# Autodesk Inventor assembly: Assembly1
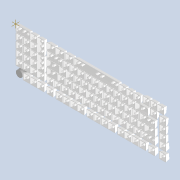
[picture p0: Inventor's stored thumbnail of the model, 180x180]
Saved by Autodesk Inventor 2021 (Build 250183000, 183)
## iProperties
Created: 2021-12-04
Part Number: Assembly1
Document SubType Name: Assembly
Designer: Matthew Flooks
Author: Matthew Flooks
## Documents named in this file (106)
- C:\Users\Matthew Flooks\Documents\GitHub\QEX103-PCB\3D Model\Assembly1.iam
- C:\Users\Matthew Flooks\Documents\GitHub\QEX103-PCB\3D Model\Layout.ipt
- C:\Users\Matthew Flooks\Documents\GitHub\QEX103-PCB\3D Model\KeyCaps\Space.ipt
- C:\Users\Matthew Flooks\Documents\GitHub\QEX103-PCB\3D Model\KeyCaps\Menu.ipt
- C:\Users\Matthew Flooks\Documents\GitHub\QEX103-PCB\3D Model\KeyCaps\CtrlRight.ipt
- C:\Users\Matthew Flooks\Documents\GitHub\QEX103-PCB\3D Model\KeyCaps\AltRight.ipt
- C:\Users\Matthew Flooks\Documents\GitHub\QEX103-PCB\3D Model\KeyCaps\Del.ipt
- C:\Users\Matthew Flooks\Documents\GitHub\QEX103-PCB\3D Model\KeyCaps\Ins.ipt
- C:\Users\Matthew Flooks\Documents\GitHub\QEX103-PCB\3D Model\KeyCaps\F12.ipt
- C:\Users\Matthew Flooks\Documents\GitHub\QEX103-PCB\3D Model\KeyCaps\F11.ipt
- C:\Users\Matthew Flooks\Documents\GitHub\QEX103-PCB\3D Model\KeyCaps\F10.ipt
- C:\Users\Matthew Flooks\Documents\GitHub\QEX103-PCB\3D Model\KeyCaps\F9.ipt
- C:\Users\Matthew Flooks\Documents\GitHub\QEX103-PCB\3D Model\KeyCaps\F8.ipt
- C:\Users\Matthew Flooks\Documents\GitHub\QEX103-PCB\3D Model\KeyCaps\F7.ipt
- C:\Users\Matthew Flooks\Documents\GitHub\QEX103-PCB\3D Model\KeyCaps\F6.ipt
- C:\Users\Matthew Flooks\Documents\GitHub\QEX103-PCB\3D Model\KeyCaps\F5.ipt
- C:\Users\Matthew Flooks\Documents\GitHub\QEX103-PCB\3D Model\KeyCaps\F4.ipt
- C:\Users\Matthew Flooks\Documents\GitHub\QEX103-PCB\3D Model\KeyCaps\F3.ipt
- C:\Users\Matthew Flooks\Documents\GitHub\QEX103-PCB\3D Model\KeyCaps\F2.ipt
- C:\Users\Matthew Flooks\Documents\GitHub\QEX103-PCB\3D Model\KeyCaps\F1.ipt
- C:\Users\Matthew Flooks\Documents\GitHub\QEX103-PCB\3D Model\KeyCaps\Prev.ipt
- C:\Users\Matthew Flooks\Documents\GitHub\QEX103-PCB\3D Model\KeyCaps\Play.ipt
- C:\Users\Matthew Flooks\Documents\GitHub\QEX103-PCB\3D Model\KeyCaps\Next.ipt
- C:\Users\Matthew Flooks\Documents\GitHub\QEX103-PCB\3D Model\KeyCaps\Esc.ipt
- C:\Users\Matthew Flooks\Documents\GitHub\QEX103-PCB\3D Model\KeyCaps\9.ipt
- C:\Users\Matthew Flooks\Documents\GitHub\QEX103-PCB\3D Model\KeyCaps\8.ipt
- C:\Users\Matthew Flooks\Documents\GitHub\QEX103-PCB\3D Model\KeyCaps\7.ipt
- C:\Users\Matthew Flooks\Documents\GitHub\QEX103-PCB\3D Model\KeyCaps\6.ipt
- C:\Users\Matthew Flooks\Documents\GitHub\QEX103-PCB\3D Model\KeyCaps\5.ipt
- C:\Users\Matthew Flooks\Documents\GitHub\QEX103-PCB\3D Model\KeyCaps\4.ipt
- C:\Users\Matthew Flooks\Documents\GitHub\QEX103-PCB\3D Model\KeyCaps\3.ipt
- C:\Users\Matthew Flooks\Documents\GitHub\QEX103-PCB\3D Model\KeyCaps\2.ipt
- C:\Users\Matthew Flooks\Documents\GitHub\QEX103-PCB\3D Model\KeyCaps\1.ipt
- C:\Users\Matthew Flooks\Documents\GitHub\QEX103-PCB\3D Model\KeyCaps\0.ipt
- C:\Users\Matthew Flooks\Documents\GitHub\QEX103-PCB\3D Model\KeyCaps\=.ipt
- C:\Users\Matthew Flooks\Documents\GitHub\QEX103-PCB\3D Model\KeyCaps\~.ipt
- C:\Users\Matthew Flooks\Documents\GitHub\QEX103-PCB\3D Model\KeyCaps\-.ipt
- C:\Users\Matthew Flooks\Documents\GitHub\QEX103-PCB\3D Model\KeyCaps\Backspace.ipt
- C:\Users\Matthew Flooks\Documents\GitHub\QEX103-PCB\3D Model\KeyCaps\Tab.ipt
- C:\Users\Matthew Flooks\Documents\GitHub\QEX103-PCB\3D Model\KeyCaps\Mod.ipt
- C:\Users\Matthew Flooks\Documents\GitHub\QEX103-PCB\3D Model\KeyCaps\ShiftRight.ipt
- C:\Users\Matthew Flooks\Documents\GitHub\QEX103-PCB\3D Model\KeyCaps\CtrlLeft.ipt
- C:\Users\Matthew Flooks\Documents\GitHub\QEX103-PCB\3D Model\KeyCaps\AltLeft.ipt
- C:\Users\Matthew Flooks\Documents\GitHub\QEX103-PCB\3D Model\KeyCaps\Win.ipt
- C:\Users\Matthew Flooks\Documents\GitHub\QEX103-PCB\3D Model\KeyCaps\BackSlash.ipt
- C:\Users\Matthew Flooks\Documents\GitHub\QEX103-PCB\3D Model\KeyCaps\Enter.ipt
- C:\Users\Matthew Flooks\Documents\GitHub\QEX103-PCB\3D Model\KeyCaps\ShiftLeft.ipt
- C:\Users\Matthew Flooks\Documents\GitHub\QEX103-PCB\3D Model\KeyCaps\,.ipt
- C:\Users\Matthew Flooks\Documents\GitHub\QEX103-PCB\3D Model\KeyCaps\..ipt
- C:\Users\Matthew Flooks\Documents\GitHub\QEX103-PCB\3D Model\KeyCaps\B.ipt
- C:\Users\Matthew Flooks\Documents\GitHub\QEX103-PCB\3D Model\KeyCaps\C.ipt
- C:\Users\Matthew Flooks\Documents\GitHub\QEX103-PCB\3D Model\KeyCaps\ForwardSlash.ipt
- C:\Users\Matthew Flooks\Documents\GitHub\QEX103-PCB\3D Model\KeyCaps\M.ipt
- C:\Users\Matthew Flooks\Documents\GitHub\QEX103-PCB\3D Model\KeyCaps\N.ipt
- C:\Users\Matthew Flooks\Documents\GitHub\QEX103-PCB\3D Model\KeyCaps\V.ipt
- C:\Users\Matthew Flooks\Documents\GitHub\QEX103-PCB\3D Model\KeyCaps\X.ipt
- C:\Users\Matthew Flooks\Documents\GitHub\QEX103-PCB\3D Model\KeyCaps\Z.ipt
- C:\Users\Matthew Flooks\Documents\GitHub\QEX103-PCB\3D Model\KeyCaps\A.ipt
- C:\Users\Matthew Flooks\Documents\GitHub\QEX103-PCB\3D Model\KeyCaps\D.ipt
- C:\Users\Matthew Flooks\Documents\GitHub\QEX103-PCB\3D Model\KeyCaps\F.ipt
- C:\Users\Matthew Flooks\Documents\GitHub\QEX103-PCB\3D Model\KeyCaps\G.ipt
- C:\Users\Matthew Flooks\Documents\GitHub\QEX103-PCB\3D Model\KeyCaps\H.ipt
- C:\Users\Matthew Flooks\Documents\GitHub\QEX103-PCB\3D Model\KeyCaps\J.ipt
- C:\Users\Matthew Flooks\Documents\GitHub\QEX103-PCB\3D Model\KeyCaps\K.ipt
- C:\Users\Matthew Flooks\Documents\GitHub\QEX103-PCB\3D Model\KeyCaps\L.ipt
- C:\Users\Matthew Flooks\Documents\GitHub\QEX103-PCB\3D Model\KeyCaps\S.ipt
- C:\Users\Matthew Flooks\Documents\GitHub\QEX103-PCB\3D Model\KeyCaps\'.ipt
- C:\Users\Matthew Flooks\Documents\GitHub\QEX103-PCB\3D Model\KeyCaps\;.ipt
- C:\Users\Matthew Flooks\Documents\GitHub\QEX103-PCB\3D Model\KeyCaps\Q.ipt
- C:\Users\Matthew Flooks\Documents\GitHub\QEX103-PCB\3D Model\KeyCaps\E.ipt
- C:\Users\Matthew Flooks\Documents\GitHub\QEX103-PCB\3D Model\KeyCaps\I.ipt
- C:\Users\Matthew Flooks\Documents\GitHub\QEX103-PCB\3D Model\KeyCaps\O.ipt
- C:\Users\Matthew Flooks\Documents\GitHub\QEX103-PCB\3D Model\KeyCaps\P.ipt
- C:\Users\Matthew Flooks\Documents\GitHub\QEX103-PCB\3D Model\KeyCaps\R.ipt
- C:\Users\Matthew Flooks\Documents\GitHub\QEX103-PCB\3D Model\KeyCaps\T.ipt
- C:\Users\Matthew Flooks\Documents\GitHub\QEX103-PCB\3D Model\KeyCaps\U.ipt
- C:\Users\Matthew Flooks\Documents\GitHub\QEX103-PCB\3D Model\KeyCaps\W.ipt
- C:\Users\Matthew Flooks\Documents\GitHub\QEX103-PCB\3D Model\KeyCaps\Y.ipt
- C:\Users\Matthew Flooks\Documents\GitHub\QEX103-PCB\3D Model\KeyCaps\[.ipt
- C:\Users\Matthew Flooks\Documents\GitHub\QEX103-PCB\3D Model\KeyCaps\].ipt
- C:\Users\Matthew Flooks\Documents\GitHub\QEX103-PCB\3D Model\KeyCaps\Home.ipt
- C:\Users\Matthew Flooks\Documents\GitHub\QEX103-PCB\3D Model\KeyCaps\End.ipt
- C:\Users\Matthew Flooks\Documents\GitHub\QEX103-PCB\3D Model\KeyCaps\PgUp.ipt
- C:\Users\Matthew Flooks\Documents\GitHub\QEX103-PCB\3D Model\KeyCaps\PgDn.ipt
- C:\Users\Matthew Flooks\Documents\GitHub\QEX103-PCB\3D Model\KeyCaps\Down.ipt
- C:\Users\Matthew Flooks\Documents\GitHub\QEX103-PCB\3D Model\KeyCaps\Left.ipt
- C:\Users\Matthew Flooks\Documents\GitHub\QEX103-PCB\3D Model\KeyCaps\Right.ipt
- C:\Users\Matthew Flooks\Documents\GitHub\QEX103-PCB\3D Model\KeyCaps\Up.ipt
- C:\Users\Matthew Flooks\Documents\GitHub\QEX103-PCB\3D Model\KeyCaps\NumEnter.ipt
- C:\Users\Matthew Flooks\Documents\GitHub\QEX103-PCB\3D Model\KeyCaps\NumPlus.ipt
- C:\Users\Matthew Flooks\Documents\GitHub\QEX103-PCB\3D Model\KeyCaps\Num0.ipt
- C:\Users\Matthew Flooks\Documents\GitHub\QEX103-PCB\3D Model\KeyCaps\Num..ipt
- C:\Users\Matthew Flooks\Documents\GitHub\QEX103-PCB\3D Model\KeyCaps\Num1.ipt
- C:\Users\Matthew Flooks\Documents\GitHub\QEX103-PCB\3D Model\KeyCaps\Num2.ipt
- C:\Users\Matthew Flooks\Documents\GitHub\QEX103-PCB\3D Model\KeyCaps\Num3.ipt
- C:\Users\Matthew Flooks\Documents\GitHub\QEX103-PCB\3D Model\KeyCaps\Num5.ipt
- C:\Users\Matthew Flooks\Documents\GitHub\QEX103-PCB\3D Model\KeyCaps\Num6.ipt
- C:\Users\Matthew Flooks\Documents\GitHub\QEX103-PCB\3D Model\KeyCaps\Num4.ipt
- C:\Users\Matthew Flooks\Documents\GitHub\QEX103-PCB\3D Model\KeyCaps\Num8.ipt
- C:\Users\Matthew Flooks\Documents\GitHub\QEX103-PCB\3D Model\KeyCaps\Num9.ipt
- C:\Users\Matthew Flooks\Documents\GitHub\QEX103-PCB\3D Model\KeyCaps\Num7.ipt
- C:\Users\Matthew Flooks\Documents\GitHub\QEX103-PCB\3D Model\KeyCaps\Num-.ipt
- C:\Users\Matthew Flooks\Documents\GitHub\QEX103-PCB\3D Model\KeyCaps\NumBackslash.ipt
- C:\Users\Matthew Flooks\Documents\GitHub\QEX103-PCB\3D Model\KeyCaps\NumLock.ipt
- C:\Users\Matthew Flooks\Documents\GitHub\QEX103-PCB\3D Model\KeyCaps\NumStar.ipt
- C:\Users\Matthew Flooks\Documents\GitHub\QEX103-PCB\3D Model\Knob.ipt
## Components (105 placed, 105 different names)
1. Layout:1 — Mate:1, Mate:2, Mate:3, Mate:4, Mate:9, Mate:10, Mate:11, Mate:12, Mate:13, Mate:14, Mate:15, Mate:16, Mate:17, Mate:18, Mate:19, Mate:20, Mate:21, Mate:22, Mate:23, Mate:24, Mate:25, Mate:26, Mate:27, Mate:28, Mate:29, Mate:30, Mate:31, Mate:32, Mate:33, Mate:34, Mate:35, Mate:36, Mate:37, Mate:38, Mate:39, Mate:40, Mate:41, Mate:42, Mate:43, Mate:44, Mate:45, Mate:46, Mate:47, Mate:48, Mate:49, Mate:50, Mate:51, Mate:52, Mate:53, Mate:54, Mate:55, Mate:56, Mate:57, Mate:58, Mate:59, Mate:60, Mate:61, Mate:62, Mate:63, Mate:64, Mate:65, Mate:66, Mate:67, Mate:68, Mate:69, Mate:70, Mate:71, Mate:72, Mate:73, Mate:74, Mate:75, Mate:76, Mate:77, Mate:78, Mate:79, Mate:80, Mate:81, Mate:82, Mate:85, Mate:86, Mate:87, Mate:88, Mate:89, Mate:90, Mate:119, Mate:120, Mate:121, Mate:122, Mate:123, Mate:124, Mate:125, Mate:126, Mate:127, Mate:128, Mate:129, Mate:130, Mate:131, Mate:132, Mate:133, Mate:134, Mate:135, Mate:136, Mate:137, Mate:138, Mate:139, Mate:140, Mate:141, Mate:142, Mate:143, Mate:144, Mate:145, Mate:146, Mate:147, Mate:148, Mate:149, Mate:150, Mate:151, Mate:152, Mate:153, Mate:154, Mate:155, Mate:156, Mate:157, Mate:158, Mate:159, Mate:160, Mate:161, Mate:162, Mate:163, Mate:164, Mate:165, Mate:166, Mate:167, Mate:168, Mate:169, Mate:170, Mate:171, Mate:172, Mate:173, Mate:174, Mate:175, Mate:176, Mate:177, Mate:178, Mate:179, Mate:180, Mate:181, Mate:182, Mate:183, Mate:184, Mate:185, Mate:186, Mate:187, Mate:188, Mate:189, Mate:190, Mate:191, Mate:192, Mate:193, Mate:194, Mate:195, Mate:196, Mate:197, Mate:198, Mate:199, Mate:200, Mate:201, Mate:202, Mate:203, Mate:204, Mate:205, Mate:206, Mate:207, Mate:208, Mate:209, Mate:210, Mate:211, Mate:212, Mate:213, Mate:214, Mate:217, Mate:218, Mate:219, Mate:220, Mate:221, Mate:222, Mate:223, Mate:224, Mate:225, Mate:226, Mate:227, Mate:228, Mate:229, Mate:230, Mate:231, Mate:232, Mate:233, Mate:234, Mate:235, Mate:236, Mate:237, Mate:238, Mate:239, Mate:240, Mate:241, Mate:242, Mate:243, Mate:244, Mate:245
2. Space:1 — Mate:3, Mate:4
3. Menu:1 — Mate:9, Mate:10
4. CtrlRight:1 — Mate:11, Mate:14
5. AltRight:1 — Mate:12, Mate:13
6. Del:1 — Mate:15, Mate:16
7. Ins:1 — Mate:17, Mate:18
8. F12:1 — Mate:19, Mate:31
9. F11:1 — Mate:20, Mate:32
10. F10:1 — Mate:21, Mate:33
11. F9:1 — Mate:22, Mate:34
12. F8:1 — Mate:23, Mate:38
13. F7:1 — Mate:24, Mate:37
14. F6:1 — Mate:25, Mate:36
15. F5:1 — Mate:26, Mate:35
16. F4:1 — Mate:27, Mate:42
17. F3:1 — Mate:28, Mate:41
18. F2:1 — Mate:29, Mate:40
19. F1:1 — Mate:30, Mate:39
20. Prev:1 — Mate:44, Mate:47
21. Play:1 — Mate:43, Mate:46
22. Next:1 — Mate:45, Mate:48
23. Esc:1 — Mate:49, Mate:50
24. 9:1 — Mate:69, Mate:70
25. 8:1 — Mate:67, Mate:68
26. 7:1 — Mate:65, Mate:66
27. 6:1 — Mate:63, Mate:64
28. 5:1 — Mate:61, Mate:62
29. 4:1 — Mate:59, Mate:60
30. 3:1 — Mate:57, Mate:58
31. 2:1 — Mate:55, Mate:56
32. 1:1 — Mate:53, Mate:54
33. 0:1 — Mate:71, Mate:72
34. =:1 — Mate:75, Mate:76
35. ~:1 — Mate:51, Mate:52
36. -:1 — Mate:73, Mate:74
37. Backspace:1 — Mate:77, Mate:78
38. Tab:1 — Mate:79, Mate:80
39. Mod:1 — Mate:81, Mate:82
40. CtrlLeft:1 — Mate:85, Mate:86
41. AltLeft:1 — Mate:89, Mate:90
42. Win:1 — Mate:87, Mate:88
43. BackSlash:1 — Mate:119, Mate:120
44. Enter:1 — Mate:121, Mate:122
45. ShiftLeft:1 — Mate:123, Mate:124
46. ,:1 — Mate:139, Mate:140
47. .:1 — Mate:141, Mate:142
48. B:1 — Mate:133, Mate:134
49. C:1 — Mate:129, Mate:130
50. ForwardSlash:1 — Mate:143, Mate:144
51. M:1 — Mate:137, Mate:138
52. N:1 — Mate:135, Mate:136
53. V:1 — Mate:131, Mate:132
54. X:1 — Mate:127, Mate:128
55. Z:1 — Mate:125, Mate:126
56. ShiftRight:1 — Mate:145, Mate:146
57. A:1 — Mate:147, Mate:148
58. D:1 — Mate:151, Mate:152
59. F:1 — Mate:153, Mate:154
60. G:1 — Mate:155, Mate:156
61. H:1 — Mate:157, Mate:158
62. J:1 — Mate:159, Mate:160
63. K:1 — Mate:161, Mate:162
64. L:1 — Mate:163, Mate:164
65. S:1 — Mate:149, Mate:150
66. ':1 — Mate:165, Mate:166
67. ;:1 — Mate:167, Mate:168
68. Q:1 — Mate:169, Mate:170
69. E:1 — Mate:172, Mate:176
70. I:1 — Mate:183, Mate:184
71. O:1 — Mate:185, Mate:186
72. P:1 — Mate:187, Mate:188
73. R:1 — Mate:173, Mate:177
74. T:1 — Mate:174, Mate:178
75. U:1 — Mate:181, Mate:182
76. W:1 — Mate:171, Mate:175
77. Y:1 — Mate:179, Mate:180
78. [:1 — Mate:189, Mate:190
79. ]:1 — Mate:191, Mate:192
80. Home:1 — Mate:193, Mate:194
81. End:1 — Mate:195, Mate:196
82. PgUp:1 — Mate:197, Mate:198
83. PgDn:1 — Mate:199, Mate:200
84. Down:1 — Mate:201, Mate:202
85. Left:1 — Mate:203, Mate:204
86. Right:1 — Mate:205, Mate:206
87. Up:1 — Mate:207, Mate:208
88. NumEnter:1 — Mate:211, Mate:212
89. NumPlus:1 — Mate:209, Mate:210
90. Num0:1 — Mate:213, Mate:214
91. Num.:1 — Mate:223, Mate:224
92. Num1:1 — Mate:221, Mate:222
93. Num2:1 — Mate:219, Mate:220
94. Num3:1 — Mate:217, Mate:218
95. Num4:1 — Mate:225, Mate:226
96. Num5:1 — Mate:229, Mate:230
97. Num6:1 — Mate:227, Mate:228
98. Num7:1 — Mate:231, Mate:232
99. Num8:1 — Mate:233, Mate:234
100. Num9:1 — Mate:235, Mate:236
101. Num-:1 — Mate:243, Mate:244
102. NumBackslash:1 — Mate:239, Mate:240
103. NumLock:1 — Mate:237, Mate:238
104. NumStar:1 — Mate:241, Mate:242
105. Knob:1 — Mate:245, Mate:246
## Relationships (210: Mate 210)
- Mate:1: Layout:1
- Mate:2: Layout:1
- Mate:3: Layout:1 ↔ Space:1
- Mate:4: Layout:1 ↔ Space:1
- Mate:9: Layout:1 ↔ Menu:1
- Mate:10: Layout:1 ↔ Menu:1
- Mate:11: Layout:1 ↔ CtrlRight:1
- Mate:12: Layout:1 ↔ AltRight:1
- Mate:13: Layout:1 ↔ AltRight:1
- Mate:14: Layout:1 ↔ CtrlRight:1
- Mate:15: Layout:1 ↔ Del:1
- Mate:16: Layout:1 ↔ Del:1
- Mate:17: Layout:1 ↔ Ins:1
- Mate:18: Layout:1 ↔ Ins:1
- Mate:19: Layout:1 ↔ F12:1
- Mate:20: Layout:1 ↔ F11:1
- Mate:21: Layout:1 ↔ F10:1
- Mate:22: Layout:1 ↔ F9:1
- Mate:23: Layout:1 ↔ F8:1
- Mate:24: Layout:1 ↔ F7:1
- Mate:25: Layout:1 ↔ F6:1
- Mate:26: Layout:1 ↔ F5:1
- Mate:27: Layout:1 ↔ F4:1
- Mate:28: Layout:1 ↔ F3:1
- Mate:29: Layout:1 ↔ F2:1
- Mate:30: Layout:1 ↔ F1:1
- Mate:31: Layout:1 ↔ F12:1
- Mate:32: Layout:1 ↔ F11:1
- Mate:33: Layout:1 ↔ F10:1
- Mate:34: Layout:1 ↔ F9:1
- Mate:35: Layout:1 ↔ F5:1
- Mate:36: Layout:1 ↔ F6:1
- Mate:37: Layout:1 ↔ F7:1
- Mate:38: Layout:1 ↔ F8:1
- Mate:39: Layout:1 ↔ F1:1
- Mate:40: Layout:1 ↔ F2:1
- Mate:41: Layout:1 ↔ F3:1
- Mate:42: Layout:1 ↔ F4:1
- Mate:43: Layout:1 ↔ Play:1
- Mate:44: Layout:1 ↔ Prev:1
- Mate:45: Layout:1 ↔ Next:1
- Mate:46: Layout:1 ↔ Play:1
- Mate:47: Layout:1 ↔ Prev:1
- Mate:48: Layout:1 ↔ Next:1
- Mate:49: Layout:1 ↔ Esc:1
- Mate:50: Layout:1 ↔ Esc:1
- Mate:51: Layout:1 ↔ ~:1
- Mate:52: Layout:1 ↔ ~:1
- Mate:53: Layout:1 ↔ 1:1
- Mate:54: Layout:1 ↔ 1:1
- Mate:55: Layout:1 ↔ 2:1
- Mate:56: Layout:1 ↔ 2:1
- Mate:57: Layout:1 ↔ 3:1
- Mate:58: Layout:1 ↔ 3:1
- Mate:59: Layout:1 ↔ 4:1
- Mate:60: Layout:1 ↔ 4:1
- Mate:61: Layout:1 ↔ 5:1
- Mate:62: Layout:1 ↔ 5:1
- Mate:63: Layout:1 ↔ 6:1
- Mate:64: Layout:1 ↔ 6:1
- Mate:65: Layout:1 ↔ 7:1
- Mate:66: Layout:1 ↔ 7:1
- Mate:67: Layout:1 ↔ 8:1
- Mate:68: Layout:1 ↔ 8:1
- Mate:69: Layout:1 ↔ 9:1
- Mate:70: Layout:1 ↔ 9:1
- Mate:71: Layout:1 ↔ 0:1
- Mate:72: Layout:1 ↔ 0:1
- Mate:73: Layout:1 ↔ -:1
- Mate:74: Layout:1 ↔ -:1
- Mate:75: Layout:1 ↔ =:1
- Mate:76: Layout:1 ↔ =:1
- Mate:77: Layout:1 ↔ Backspace:1
- Mate:78: Layout:1 ↔ Backspace:1
- Mate:79: Layout:1 ↔ Tab:1
- Mate:80: Layout:1 ↔ Tab:1
- Mate:81: Layout:1 ↔ Mod:1
- Mate:82: Layout:1 ↔ Mod:1
- Mate:85: Layout:1 ↔ CtrlLeft:1
- Mate:86: Layout:1 ↔ CtrlLeft:1
- Mate:87: Layout:1 ↔ Win:1
- Mate:88: Layout:1 ↔ Win:1
- Mate:89: Layout:1 ↔ AltLeft:1
- Mate:90: Layout:1 ↔ AltLeft:1
- Mate:119: Layout:1 ↔ BackSlash:1
- Mate:120: Layout:1 ↔ BackSlash:1
- Mate:121: Layout:1 ↔ Enter:1
- Mate:122: Layout:1 ↔ Enter:1
- Mate:123: Layout:1 ↔ ShiftLeft:1
- Mate:124: Layout:1 ↔ ShiftLeft:1
- Mate:125: Layout:1 ↔ Z:1
- Mate:126: Layout:1 ↔ Z:1
- Mate:127: Layout:1 ↔ X:1
- Mate:128: Layout:1 ↔ X:1
- Mate:129: Layout:1 ↔ C:1
- Mate:130: Layout:1 ↔ C:1
- Mate:131: Layout:1 ↔ V:1
- Mate:132: Layout:1 ↔ V:1
- Mate:133: Layout:1 ↔ B:1
- Mate:134: Layout:1 ↔ B:1
- Mate:135: Layout:1 ↔ N:1
- Mate:136: Layout:1 ↔ N:1
- Mate:137: Layout:1 ↔ M:1
- Mate:138: Layout:1 ↔ M:1
- Mate:139: Layout:1 ↔ ,:1
- Mate:140: Layout:1 ↔ ,:1
- Mate:141: Layout:1 ↔ .:1
- Mate:142: Layout:1 ↔ .:1
- Mate:143: Layout:1 ↔ ForwardSlash:1
- Mate:144: Layout:1 ↔ ForwardSlash:1
- Mate:145: Layout:1 ↔ ShiftRight:1
- Mate:146: Layout:1 ↔ ShiftRight:1
- Mate:147: Layout:1 ↔ A:1
- Mate:148: Layout:1 ↔ A:1
- Mate:149: Layout:1 ↔ S:1
- Mate:150: Layout:1 ↔ S:1
- Mate:151: Layout:1 ↔ D:1
- Mate:152: Layout:1 ↔ D:1
- Mate:153: Layout:1 ↔ F:1
- Mate:154: Layout:1 ↔ F:1
- Mate:155: Layout:1 ↔ G:1
- Mate:156: Layout:1 ↔ G:1
- Mate:157: Layout:1 ↔ H:1
- Mate:158: Layout:1 ↔ H:1
- Mate:159: Layout:1 ↔ J:1
- Mate:160: Layout:1 ↔ J:1
- Mate:161: Layout:1 ↔ K:1
- Mate:162: Layout:1 ↔ K:1
- Mate:163: Layout:1 ↔ L:1
- Mate:164: Layout:1 ↔ L:1
- Mate:165: Layout:1 ↔ ':1
- Mate:166: Layout:1 ↔ ':1
- Mate:167: Layout:1 ↔ ;:1
- Mate:168: Layout:1 ↔ ;:1
- Mate:169: Layout:1 ↔ Q:1
- Mate:170: Layout:1 ↔ Q:1
- Mate:171: Layout:1 ↔ W:1
- Mate:172: Layout:1 ↔ E:1
- Mate:173: Layout:1 ↔ R:1
- Mate:174: Layout:1 ↔ T:1
- Mate:175: Layout:1 ↔ W:1
- Mate:176: Layout:1 ↔ E:1
- Mate:177: Layout:1 ↔ R:1
- Mate:178: Layout:1 ↔ T:1
- Mate:179: Layout:1 ↔ Y:1
- Mate:180: Layout:1 ↔ Y:1
- Mate:181: Layout:1 ↔ U:1
- Mate:182: Layout:1 ↔ U:1
- Mate:183: Layout:1 ↔ I:1
- Mate:184: Layout:1 ↔ I:1
- Mate:185: Layout:1 ↔ O:1
- Mate:186: Layout:1 ↔ O:1
- Mate:187: Layout:1 ↔ P:1
- Mate:188: Layout:1 ↔ P:1
- Mate:189: Layout:1 ↔ [:1
- Mate:190: Layout:1 ↔ [:1
- Mate:191: Layout:1 ↔ ]:1
- Mate:192: Layout:1 ↔ ]:1
- Mate:193: Layout:1 ↔ Home:1
- Mate:194: Layout:1 ↔ Home:1
- Mate:195: Layout:1 ↔ End:1
- Mate:196: Layout:1 ↔ End:1
- Mate:197: Layout:1 ↔ PgUp:1
- Mate:198: Layout:1 ↔ PgUp:1
- Mate:199: Layout:1 ↔ PgDn:1
- Mate:200: Layout:1 ↔ PgDn:1
- Mate:201: Layout:1 ↔ Down:1
- Mate:202: Layout:1 ↔ Down:1
- Mate:203: Layout:1 ↔ Left:1
- Mate:204: Layout:1 ↔ Left:1
- Mate:205: Layout:1 ↔ Right:1
- Mate:206: Layout:1 ↔ Right:1
- Mate:207: Layout:1 ↔ Up:1
- Mate:208: Layout:1 ↔ Up:1
- Mate:209: Layout:1 ↔ NumPlus:1
- Mate:210: Layout:1 ↔ NumPlus:1
- Mate:211: Layout:1 ↔ NumEnter:1
- Mate:212: Layout:1 ↔ NumEnter:1
- Mate:213: Layout:1 ↔ Num0:1
- Mate:214: Layout:1 ↔ Num0:1
- Mate:217: Layout:1 ↔ Num3:1
- Mate:218: Layout:1 ↔ Num3:1
- Mate:219: Layout:1 ↔ Num2:1
- Mate:220: Layout:1 ↔ Num2:1
- Mate:221: Layout:1 ↔ Num1:1
- Mate:222: Layout:1 ↔ Num1:1
- Mate:223: Layout:1 ↔ Num.:1
- Mate:224: Layout:1 ↔ Num.:1
- Mate:225: Layout:1 ↔ Num4:1
- Mate:226: Layout:1 ↔ Num4:1
- Mate:227: Layout:1 ↔ Num6:1
- Mate:228: Layout:1 ↔ Num6:1
- Mate:229: Layout:1 ↔ Num5:1
- Mate:230: Layout:1 ↔ Num5:1
- Mate:231: Layout:1 ↔ Num7:1
- Mate:232: Layout:1 ↔ Num7:1
- Mate:233: Layout:1 ↔ Num8:1
- Mate:234: Layout:1 ↔ Num8:1
- Mate:235: Layout:1 ↔ Num9:1
- Mate:236: Layout:1 ↔ Num9:1
- Mate:237: Layout:1 ↔ NumLock:1
- Mate:238: Layout:1 ↔ NumLock:1
- Mate:239: Layout:1 ↔ NumBackslash:1
- Mate:240: Layout:1 ↔ NumBackslash:1
- Mate:241: Layout:1 ↔ NumStar:1
- Mate:242: Layout:1 ↔ NumStar:1
- Mate:243: Layout:1 ↔ Num-:1
- Mate:244: Layout:1 ↔ Num-:1
- Mate:245: Layout:1 ↔ Knob:1
- Mate:246: Knob:1
